# Autodesk Inventor assembly: Contrapeso
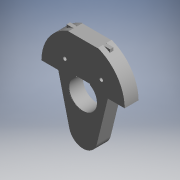
[picture p0: Inventor's stored thumbnail of the model, 180x180]
Saved by Autodesk Inventor 2019.3 (Build 233278000, 278)
## iProperties
Part Number: Contrapeso
Document SubType Name: Assembly
Designer: Usuario
Author: Usuario
## Documents named in this file (3)
- C:\Users\Usuario\Documents\6 semestre\Dinámica\Proyecto2\Propio\Contrapeso.iam
- C:\Users\Usuario\Documents\6 semestre\Dinámica\Proyecto2\Propio\Ajuste.ipt
- C:\Users\Usuario\Documents\6 semestre\Dinámica\Proyecto2\Propio\Contrap.ipt
## Components (2 placed, 2 different names)
1. Ajuste:1 — Rigid:1
2. Contrap:1 — Rigid:1
## Relationships (1: WeldJoint 1)
- Rigid:1 [WeldJoint]: Ajuste:1 ↔ Contrap:1
